# Autodesk Inventor assembly: mini sand
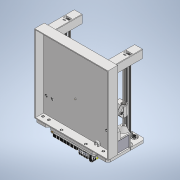
[picture p0: Inventor's stored thumbnail of the model, 180x180]
Saved by Autodesk Inventor 2022 (Build 260153000, 153)
## iProperties
Created: 2022-04-23
Part Number: mini sand
Document SubType Name: Assembly
Designer: Administrator
Title: mini sand v11
Author: Administrator
## Documents named in this file (31)
- Y:\Projects\Mini_Sand_Table\Mini Sand Table.iam
- Y:\Projects\Mini_Sand_Table\Hardware\Linear Rods\4mm x 140mm Rod.ipt
- Y:\Projects\Mini_Sand_Table\Hardware\Bearings\603ZZ Roller Bearing.ipt
- Y:\Projects\Mini_Sand_Table\Hardware\Linear Rods\4mm x 130mm Rod.ipt
- Y:\Projects\Mini_Sand_Table\Hardware\GT2 16T Pulley.ipt
- Y:\Projects\Mini_Sand_Table\Hardware\Magnet.ipt
- Y:\Projects\Mini_Sand_Table\Hardware\Bearings\LM4UU.ipt
- Y:\Projects\Mini_Sand_Table\3D Printed\Table Top.ipt
- Y:\Projects\Mini_Sand_Table\Electronics\NEMA 11.ipt
- Y:\Projects\Mini_Sand_Table\3D Printed\Belt Retainer.ipt
- Y:\Projects\Mini_Sand_Table\3D Printed\Magnet Mount Lower.ipt
- Y:\Projects\Mini_Sand_Table\3D Printed\Models with Heat Set Inserts\XY Joiner HSI.iam
- Y:\Projects\Mini_Sand_Table\3D Printed\Models with Heat Set Inserts\Idle Bearing Mount HSI.iam
- Y:\Projects\Mini_Sand_Table\Hardware\M3\Nuts\M3 Hex Nut.ipt
- Y:\Projects\Mini_Sand_Table\Hardware\4mm Ball.ipt
- Y:\Projects\Mini_Sand_Table\Electronics\SKR Mini E3 v3.0.ipt
- Y:\Projects\Mini_Sand_Table\3D Printed\Sand Cover.ipt
- Y:\Projects\Mini_Sand_Table\3D Printed\Models with Heat Set Inserts\Magnet Mount HSI.iam
- Y:\Projects\Mini_Sand_Table\3D Printed\Models with Heat Set Inserts\Motor Mount HSI.iam
- Y:\Projects\Mini_Sand_Table\3D Printed\Models with Heat Set Inserts\Driver Board Mount HSI.iam
- Y:\Projects\Mini_Sand_Table\Hardware\M2.5\M2.5 x 10 mm SHCS.ipt
- Y:\Projects\Mini_Sand_Table\Hardware\M2.5\M2.5 x 6 mm SHCS.ipt
- Y:\Projects\Mini_Sand_Table\Hardware\M3\Bolts\M3 x 16 mm FHCS.ipt
- Y:\Projects\Mini_Sand_Table\Hardware\M3\Bolts\M3 x 10 mm FHCS.ipt
- Y:\Projects\Mini_Sand_Table\Electronics\DC Jack.ipt
- Y:\Projects\Mini_Sand_Table\Electronics\DC Jack Nut.ipt
- Y:\Projects\Mini_Sand_Table\Hardware\M3\Nuts\5mm M3 Brass Standoff.ipt
- Y:\Projects\Mini_Sand_Table\Hardware\M3\Bolts\M3 x 6 mm FHCS.ipt
- Y:\Projects\Mini_Sand_Table\Electronics\Led Tape.ipt
- Y:\Projects\Mini_Sand_Table\Hardware\GT2 Belt.ipt
- Y:\Projects\Mini_Sand_Table\3D Printed\Belt Clip.ipt
## Components (94 placed, 32 different names)
1. Led Tape:1 — Mate:51, Flush:4, Mate:52
2. GT2 Belt:1 — Mate:53
3. Belt Clip:1 — Mate:53, Mate:54, Flush:5, Insert:253
4. 5mm M3 Brass Standoff:5 — Insert:225
5. 5mm M3 Brass Standoff:4 — Insert:226
6. 5mm M3 Brass Standoff:3 — Insert:229
7. 5mm M3 Brass Standoff:2 — Insert:227
8. 5mm M3 Brass Standoff:1 — Insert:228
9. magnet:1 — Mate:31, Insert:107
10. 4mm x 140mm Rod:1 — Insert:60, Mate:46
11. 4mm x 140mm Rod:2 — Mate:9, Insert:61
12. 4mm x 130mm Rod:2 — Insert:95, Mate:43, Mate:45
13. 4mm x 130mm Rod:3 — Insert:87, Mate:44, Mate:49
14. GT2 16T Pulley:2 — Insert:68
15. gt2 pulley 16t v1:1 — Insert:65
16. 4mm Ball:1 — Mate:31, Tangent:1
17. Belt Retainer:2 — Insert:194, Insert:195
18. XY Joiner HSI:3 [sub-assembly] — Mate:44, Mate:45, Insert:202, Insert:232, Insert:233, Angle:1, Angle:2
19. Magnet Mount Lower:1 — Insert:159, Insert:230, Insert:231, Flush:3, Mate:54, Flush:5
20. Magnet Mount HSI:1 [sub-assembly] — Insert:107, Insert:230, Insert:231, Mate:50
21. Motor Mount HSI:1 [sub-assembly] — Insert:108, Insert:109, Insert:110, Insert:111, Insert:146, Insert:147
22. Motor Mount HSI:2 [sub-assembly] — Insert:112, Insert:113, Insert:114, Insert:148, Insert:149
23. table mount (1):1 [sub-assembly] — Insert:56, Insert:57, Insert:60, Insert:90, Insert:236, Angle:5, Insert:252
24. table mount (1):2 [sub-assembly] — Insert:58, Insert:59, Insert:61, Insert:89, Insert:237, Angle:6, Insert:251
25. XY Joiner HSI:2 [sub-assembly] — Insert:80, Insert:81, Insert:87, Insert:95, Insert:98, Insert:99, Insert:173, Insert:203, Insert:234, Insert:235, Angle:3, Angle:4
26. Belt Retainer:1 — Insert:82, Insert:83, Insert:198, Insert:199
27. Table Top:1 — Insert:56, Insert:57, Insert:58, Insert:59, Tangent:1, Mate:39, Mate:40, Mate:41, Insert:108, Insert:109, Insert:112, Insert:113, Insert:115, Insert:116, Insert:212, Insert:213, Insert:217, Insert:218, Insert:219, Insert:220, Insert:221, Insert:222, Insert:223, Insert:224, Insert:245, Insert:246, Insert:247, Insert:248, Insert:249, Insert:250
28. Driver Board Mount HSI:1 [sub-assembly] — Insert:115, Insert:116, Insert:142, Insert:143, Insert:144, Insert:145, Mate:47, Insert:200, Insert:201, Flush:1, Mate:48, Flush:2, Insert:225, Insert:226, Insert:227, Insert:228, Insert:229
29. Sand Cover:1 — Mate:39, Mate:40, Mate:41, Mate:51, Flush:4, Mate:52
30. DC Jack:1 — Insert:200
31. DC Jack Nut:1 — Insert:201
32. NEMA 11:1 — Insert:68, Insert:114, Mate:47
33. NEMA 11:2 — Insert:65, Insert:110, Insert:111
34. SKR Mini E3 v3.0:2 — Flush:1, Mate:48, Flush:2, Insert:240, Insert:241, Insert:242, Insert:243, Insert:244
35. LM4UU:3 — Mate:9, Insert:98
36. LM4UU:4 — Insert:99
37. LM4UU:5 — Insert:159, Mate:43
38. LM4UU:6 — Flush:3, Mate:49, Mate:50
39. LM4UU:7 — Mate:46
40. LM4UU:8
41. 603ZZ Roller Bearing:5 — Insert:81, Insert:82
42. 603ZZ Roller Bearing:6 — Insert:80, Insert:83
43. 603ZZ Roller Bearing:7
44. 603ZZ Roller Bearing:8
45. roller bearing:3 — Insert:90
46. roller bearing:4 — Insert:89
47. M3 Hex Nut:3 — Insert:236, Angle:5
48. M3 Hex Nut:4 — Insert:237, Angle:6
49. M3 Hex Nut:8 — Insert:232, Angle:2
50. M3 Hex Nut:7 — Insert:233, Angle:1
51. M3 Hex Nut:2 — Insert:234, Angle:4
52. M3 Hex Nut:6 — Insert:235, Angle:3
53. M3 x 6 mm FHCS:6 — Insert:248
54. M3 x 6 mm FHCS:5 — Insert:247
55. M3 x 6 mm FHCS:4 — Insert:250
56. M3 x 6 mm FHCS:3 — Insert:249
57. M3 x 6 mm FHCS:2 — Insert:246
58. M3 x 6 mm FHCS:1 — Insert:245
59. M3 x 6 mm FHCS:5 — Insert:244
60. M3 x 6 mm FHCS:4 — Insert:241
61. M3 x 6 mm FHCS:3 — Insert:242
62. M3 x 6 mm FHCS:2 — Insert:243
63. M3 x 6 mm FHCS:1 — Insert:240
64. M3 x 10 mm FHCS:25 — Insert:222
65. M3 x 10 mm FHCS:24 — Insert:224
66. M3 x 10 mm FHCS:23 — Insert:223
67. M3 x 10 mm FHCS:7 — Insert:219
68. M3 x 10 mm FHCS:8 — Insert:212
69. M3 x 10 mm FHCS:9 — Insert:221
70. M3 x 10 mm FHCS:10 — Insert:213
71. M3 x 10 mm FHCS:11 — Insert:220
72. M3 x 10 mm FHCS:12 — Insert:217
73. M3 x 10 mm FHCS:15 — Insert:218
74. M3 x 10 mm FHCS:6 — Insert:199
75. M3 x 10 mm FHCS:5 — Insert:198
76. M3 x 10 mm FHCS:4
77. M3 x 10 mm FHCS:3
78. M3 x 10 mm FHCS:2 — Insert:195
79. M3 x 10 mm FHCS:1 — Insert:194
80. M3 x 16 mm FHCS:7 — Insert:253
81. M3 x 16 mm FHCS:6 — Insert:251
82. M3 x 16 mm FHCS:5 — Insert:252
83. M3 x 16 mm FHCS:1 — Insert:173
84. M3 x 16 mm FHCS:2 — Insert:203
85. M3 x 16 mm FHCS:3
86. M3 x 16 mm FHCS:4 — Insert:202
87. M2.5 x 10 mm SHCS:1 — Insert:143
88. M2.5 x 10 mm SHCS:2 — Insert:142
89. M2.5 x 10 mm SHCS:3 — Insert:145
90. M2.5 x 10 mm SHCS:4 — Insert:144
91. M2.5 x 6 mm SHCS:1 — Insert:146
92. M2.5 x 6 mm SHCS:2 — Insert:147
93. M2.5 x 6 mm SHCS:3 — Insert:148
94. M2.5 x 6 mm SHCS:4 — Insert:149
## Relationships (119: Insert 90, Mate 17, Angle 6, Flush 5, Tangent 1)
- Mate:9: 4mm x 140mm Rod:2 ↔ LM4UU:3
- Insert:56: table mount (1):1 ↔ Table Top:1
- Insert:57: table mount (1):1 ↔ Table Top:1
- Insert:58: table mount (1):2 ↔ Table Top:1
- Insert:59: table mount (1):2 ↔ Table Top:1
- Insert:60: 4mm x 140mm Rod:1 ↔ table mount (1):1
- Insert:61: 4mm x 140mm Rod:2 ↔ table mount (1):2
- Insert:65: gt2 pulley 16t v1:1 ↔ NEMA 11:2
- Insert:68: GT2 16T Pulley:2 ↔ NEMA 11:1
- Insert:80: XY Joiner HSI:2 ↔ 603ZZ Roller Bearing:6
- Insert:81: XY Joiner HSI:2 ↔ 603ZZ Roller Bearing:5
- Insert:82: Belt Retainer:1 ↔ 603ZZ Roller Bearing:5
- Insert:83: Belt Retainer:1 ↔ 603ZZ Roller Bearing:6
- Insert:87: 4mm x 130mm Rod:3 ↔ XY Joiner HSI:2
- Insert:89: table mount (1):2 ↔ roller bearing:4
- Insert:90: table mount (1):1 ↔ roller bearing:3
- Insert:95: 4mm x 130mm Rod:2 ↔ XY Joiner HSI:2
- Insert:98: XY Joiner HSI:2 ↔ LM4UU:3
- Insert:99: XY Joiner HSI:2 ↔ LM4UU:4
- Mate:31: magnet:1 ↔ 4mm Ball:1
- Tangent:1: 4mm Ball:1 ↔ Table Top:1
- Mate:39: Table Top:1 ↔ Sand Cover:1
- Mate:40: Table Top:1 ↔ Sand Cover:1
- Mate:41: Table Top:1 ↔ Sand Cover:1
- Insert:107: magnet:1 ↔ Magnet Mount HSI:1
- Insert:108: Motor Mount HSI:1 ↔ Table Top:1
- Insert:109: Motor Mount HSI:1 ↔ Table Top:1
- Insert:110: Motor Mount HSI:1 ↔ NEMA 11:2
- Insert:111: Motor Mount HSI:1 ↔ NEMA 11:2
- Insert:112: Motor Mount HSI:2 ↔ Table Top:1
- Insert:113: Motor Mount HSI:2 ↔ Table Top:1
- Insert:114: Motor Mount HSI:2 ↔ NEMA 11:1
- Insert:115: Table Top:1 ↔ Driver Board Mount HSI:1
- Insert:116: Table Top:1 ↔ Driver Board Mount HSI:1
- Insert:142: Driver Board Mount HSI:1 ↔ M2.5 x 10 mm SHCS:2
- Insert:143: Driver Board Mount HSI:1 ↔ M2.5 x 10 mm SHCS:1
- Insert:144: Driver Board Mount HSI:1 ↔ M2.5 x 10 mm SHCS:4
- Insert:145: Driver Board Mount HSI:1 ↔ M2.5 x 10 mm SHCS:3
- Insert:146: Motor Mount HSI:1 ↔ M2.5 x 6 mm SHCS:1
- Insert:147: Motor Mount HSI:1 ↔ M2.5 x 6 mm SHCS:2
- Insert:148: Motor Mount HSI:2 ↔ M2.5 x 6 mm SHCS:3
- Insert:149: Motor Mount HSI:2 ↔ M2.5 x 6 mm SHCS:4
- Insert:159: Magnet Mount Lower:1 ↔ LM4UU:5
- Mate:43: 4mm x 130mm Rod:2 ↔ LM4UU:5
- Insert:173: XY Joiner HSI:2 ↔ M3 x 16 mm FHCS:1
- [Insert]: XY Joiner HSI:3 ↔ 603ZZ Roller Bearing:8
- [Insert]: XY Joiner HSI:3 ↔ 603ZZ Roller Bearing:7
- [Insert]: Belt Retainer:2 ↔ 603ZZ Roller Bearing:7
- [Insert]: Belt Retainer:2 ↔ 603ZZ Roller Bearing:8
- [Insert]: XY Joiner HSI:3 ↔ LM4UU:7
- [Insert]: XY Joiner HSI:3 ↔ LM4UU:8
- [Insert]: XY Joiner HSI:3 ↔ M3 x 16 mm FHCS:3
- Mate:44: 4mm x 130mm Rod:3 ↔ XY Joiner HSI:3
- Mate:45: 4mm x 130mm Rod:2 ↔ XY Joiner HSI:3
- Mate:46: 4mm x 140mm Rod:1 ↔ LM4UU:7
- Mate:47: Driver Board Mount HSI:1 ↔ NEMA 11:1
- Insert:194: Belt Retainer:2 ↔ M3 x 10 mm FHCS:1
- Insert:195: Belt Retainer:2 ↔ M3 x 10 mm FHCS:2
- Insert:198: Belt Retainer:1 ↔ M3 x 10 mm FHCS:5
- Insert:199: Belt Retainer:1 ↔ M3 x 10 mm FHCS:6
- Insert:200: Driver Board Mount HSI:1 ↔ DC Jack:1
- Insert:201: Driver Board Mount HSI:1 ↔ DC Jack Nut:1
- Insert:202: XY Joiner HSI:3 ↔ M3 x 16 mm FHCS:4
- Insert:203: XY Joiner HSI:2 ↔ M3 x 16 mm FHCS:2
- Insert:212: Table Top:1 ↔ M3 x 10 mm FHCS:8
- Insert:213: Table Top:1 ↔ M3 x 10 mm FHCS:10
- Insert:217: Table Top:1 ↔ M3 x 10 mm FHCS:12
- Insert:218: Table Top:1 ↔ M3 x 10 mm FHCS:15
- Insert:219: Table Top:1 ↔ M3 x 10 mm FHCS:7
- Insert:220: Table Top:1 ↔ M3 x 10 mm FHCS:11
- Insert:221: Table Top:1 ↔ M3 x 10 mm FHCS:9
- Flush:1 (2 mm): Driver Board Mount HSI:1 ↔ SKR Mini E3 v3.0:2
- Mate:48 (5 mm): Driver Board Mount HSI:1 ↔ SKR Mini E3 v3.0:2
- Flush:2 (3.35 mm): Driver Board Mount HSI:1 ↔ SKR Mini E3 v3.0:2
- Insert:222: Table Top:1 ↔ M3 x 10 mm FHCS:25
- Insert:223: Table Top:1 ↔ M3 x 10 mm FHCS:23
- Insert:224: Table Top:1 ↔ M3 x 10 mm FHCS:24
- Insert:225: 5mm M3 Brass Standoff:5 ↔ Driver Board Mount HSI:1
- Insert:226: 5mm M3 Brass Standoff:4 ↔ Driver Board Mount HSI:1
- Insert:227: 5mm M3 Brass Standoff:2 ↔ Driver Board Mount HSI:1
- Insert:228: 5mm M3 Brass Standoff:1 ↔ Driver Board Mount HSI:1
- Insert:229: 5mm M3 Brass Standoff:3 ↔ Driver Board Mount HSI:1
- Insert:230: Magnet Mount Lower:1 ↔ Magnet Mount HSI:1
- Insert:231: Magnet Mount Lower:1 ↔ Magnet Mount HSI:1
- Flush:3: Magnet Mount Lower:1 ↔ LM4UU:6
- Mate:49: 4mm x 130mm Rod:3 ↔ LM4UU:6
- Mate:50 (0.5 mm): Magnet Mount HSI:1 ↔ LM4UU:6
- Insert:232: XY Joiner HSI:3 ↔ M3 Hex Nut:8
- Insert:233: XY Joiner HSI:3 ↔ M3 Hex Nut:7
- Angle:1 (0 deg): XY Joiner HSI:3 ↔ M3 Hex Nut:7
- Angle:2 (0 deg): XY Joiner HSI:3 ↔ M3 Hex Nut:8
- Insert:234: XY Joiner HSI:2 ↔ M3 Hex Nut:2
- Insert:235: XY Joiner HSI:2 ↔ M3 Hex Nut:6
- Angle:3 (0 deg): XY Joiner HSI:2 ↔ M3 Hex Nut:6
- Angle:4 (0 deg): XY Joiner HSI:2 ↔ M3 Hex Nut:2
- Insert:236: table mount (1):1 ↔ M3 Hex Nut:3
- Angle:5 (0 deg): table mount (1):1 ↔ M3 Hex Nut:3
- Insert:237: table mount (1):2 ↔ M3 Hex Nut:4
- Angle:6 (0 deg): table mount (1):2 ↔ M3 Hex Nut:4
- Insert:240: SKR Mini E3 v3.0:2 ↔ M3 x 6 mm FHCS:1
- Insert:241: SKR Mini E3 v3.0:2 ↔ M3 x 6 mm FHCS:4
- Insert:242: SKR Mini E3 v3.0:2 ↔ M3 x 6 mm FHCS:3
- Insert:243: SKR Mini E3 v3.0:2 ↔ M3 x 6 mm FHCS:2
- Insert:244: SKR Mini E3 v3.0:2 ↔ M3 x 6 mm FHCS:5
- Insert:245: Table Top:1 ↔ M3 x 6 mm FHCS:1
- Insert:246: Table Top:1 ↔ M3 x 6 mm FHCS:2
- Insert:247: Table Top:1 ↔ M3 x 6 mm FHCS:5
- Insert:248: Table Top:1 ↔ M3 x 6 mm FHCS:6
- Insert:249: Table Top:1 ↔ M3 x 6 mm FHCS:3
- Insert:250: Table Top:1 ↔ M3 x 6 mm FHCS:4
- Insert:251: table mount (1):2 ↔ M3 x 16 mm FHCS:6
- Insert:252: table mount (1):1 ↔ M3 x 16 mm FHCS:5
- Mate:51: Led Tape:1 ↔ Sand Cover:1
- Flush:4: Led Tape:1 ↔ Sand Cover:1
- Mate:52: Led Tape:1 ↔ Sand Cover:1
- Mate:53: GT2 Belt:1 ↔ Belt Clip:1
- Mate:54: Belt Clip:1 ↔ Magnet Mount Lower:1
- Flush:5: Belt Clip:1 ↔ Magnet Mount Lower:1
- Insert:253: Belt Clip:1 ↔ M3 x 16 mm FHCS:7
## Named parameters: d265_d159 = 0 mm, d266_d160 = 0 mm, d267_d131 = 0 mm, d268_d132 = 0 mm, d269_d133 = 0 mm, d270_d134 = 0 mm, d275_d261 = 0 mm
